# Autodesk Inventor assembly: Robot
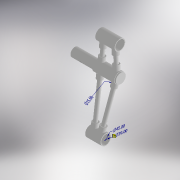
[picture p0: Inventor's stored thumbnail of the model, 180x180]
Saved by Autodesk Inventor 2021 (Build 250183000, 183)
## iProperties
Created: 2024-02-19
Part Number: Robot
Document SubType Name: Assembly
Designer: Martin
Author: Martin
## Documents named in this file (9)
- C:\Users\ASUS\OneDrive - Universidad de Antioquia\2024-1\Robótica\CAD\Robot.iam
- C:\Users\ASUS\OneDrive - Universidad de Antioquia\2024-1\Robótica\CAD\JuntaRodilla.ipt
- C:\Users\ASUS\OneDrive - Universidad de Antioquia\2024-1\Robótica\CAD\SoporteMotor.ipt
- C:\Users\ASUS\OneDrive - Universidad de Antioquia\2024-1\Robótica\CAD\Tubo1.ipt
- C:\Users\ASUS\OneDrive - Universidad de Antioquia\2024-1\Robótica\CAD\Tubo2.ipt
- C:\Users\ASUS\OneDrive - Universidad de Antioquia\2024-1\Robótica\CAD\Tubo3.ipt
- C:\Users\ASUS\OneDrive - Universidad de Antioquia\2024-1\Robótica\CAD\Tubo4.ipt
- C:\Users\ASUS\OneDrive - Universidad de Antioquia\2024-1\Robótica\CAD\JuntaRodilla2.ipt
- C:\Users\ASUS\OneDrive - Universidad de Antioquia\2024-1\Robótica\CAD\EjeRodilla3.ipt
## Components (8 placed, 8 different names)
1. JuntaRodilla:1 — Mate:5, Mate:6, Mate:11, Mate:12, Mate:13, Mate:14, Mate:17, Mate:18
2. SoporteMotor:1 — Mate:1, Mate:2, Mate:3, Mate:4
3. Tubo1:1 — Mate:1, Mate:2, Mate:5
4. Tubo2:1 — Mate:3, Mate:4, Mate:6
5. Tubo3:1 — Mate:11, Mate:12, Mate:15
6. Tubo4:1 — Mate:13, Mate:14, Mate:16
7. JuntaRodilla2:1 — Mate:15, Mate:16
8. EjeRodilla3:1 — Mate:17, Mate:18
## Relationships (14: Mate 14)
- Mate:1: SoporteMotor:1 ↔ Tubo1:1
- Mate:2 (-20 mm): SoporteMotor:1 ↔ Tubo1:1
- Mate:3: SoporteMotor:1 ↔ Tubo2:1
- Mate:4 (-20 mm): SoporteMotor:1 ↔ Tubo2:1
- Mate:5: JuntaRodilla:1 ↔ Tubo1:1
- Mate:6: JuntaRodilla:1 ↔ Tubo2:1
- Mate:11: JuntaRodilla:1 ↔ Tubo3:1
- Mate:12 (-15 mm): JuntaRodilla:1 ↔ Tubo3:1
- Mate:13: JuntaRodilla:1 ↔ Tubo4:1
- Mate:14 (-15 mm): JuntaRodilla:1 ↔ Tubo4:1
- Mate:15: Tubo3:1 ↔ JuntaRodilla2:1
- Mate:16: Tubo4:1 ↔ JuntaRodilla2:1
- Mate:17: JuntaRodilla:1 ↔ EjeRodilla3:1
- Mate:18: JuntaRodilla:1 ↔ EjeRodilla3:1
